# Autodesk Inventor assembly: top
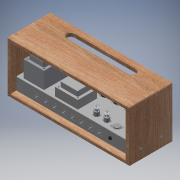
[picture p0: Inventor's stored thumbnail of the model, 180x180]
Saved by Autodesk Inventor 2016 (Build 200138000, 138)
## iProperties
Created: 2015-10-24
Part Number: top
Document SubType Name: Assembly
Designer: jeremyhale
Author: jeremyhale
## Documents named in this file (11)
- \\psf\Home\Documents\Poorhouse\git\p0001\top.iam
- \\psf\Home\Documents\Poorhouse\git\p0001\cabinet.iam
- \\psf\Home\Documents\Poorhouse\git\p0001\chassis.iam
- chassis.iam
- \\psf\Home\Documents\Poorhouse\git\p0001\cabinet-bottom.ipt
- \\psf\Home\Documents\Poorhouse\git\p0001\top\Design Accelerator\Bolted Connection6.iam
- \\psf\Home\Documents\Poorhouse\git\p0001\top\Design Accelerator\Bolted Connection7.iam
- \\psf\Home\Documents\Poorhouse\git\p0001\top\Design Accelerator\Bolted Connection8.iam
- \\psf\Home\Documents\Poorhouse\git\p0001\top\Design Accelerator\Bolted Connection9.iam
- \\psf\Home\Documents\Poorhouse\git\p0001\top\Design Accelerator\Bolted Connection10.iam
- \\psf\Home\Documents\Poorhouse\git\p0001\top\Design Accelerator\Bolted Connection11.iam
## Components (9 placed, 4 different names)
1. cabinet:1 [sub-assembly] — Flush:2, Flush:3, Flush:6, Flush:8, Flush:9, Mate:14, Mate:19, Mate:21
2. chassis:1 [sub-assembly] — Mate:1, Flush:4, Flush:5, Mate:20, Mate:22, Mate:24, Mate:26, Mate:28, Mate:30
3. cabinet-bottom:1 — Mate:1, Flush:4, Flush:5, Flush:6, Flush:8, Flush:9, Mate:14, Mate:23, Mate:25, Mate:27, Mate:29
4. Bolted Connection:5 [sub-assembly] — Mate:19, Mate:20
5. Bolted Connection:6 [sub-assembly] — Mate:21, Mate:22
6. Bolted Connection:1 [sub-assembly] — Mate:27, Mate:28
7. Bolted Connection:2 [sub-assembly] — Mate:29, Mate:30
8. Bolted Connection:3 [sub-assembly] — Mate:25, Mate:26
9. Bolted Connection:4 [sub-assembly] — Mate:23, Mate:24
## Relationships (21: Mate 14, Flush 7)
- Flush:2: cabinet:1
- Flush:3: cabinet:1
- Mate:1: chassis:1 ↔ cabinet-bottom:1
- Flush:4 (-25.4 mm): chassis:1 ↔ cabinet-bottom:1
- Flush:5: chassis:1 ↔ cabinet-bottom:1
- Flush:6: cabinet:1 ↔ cabinet-bottom:1
- Flush:8: cabinet:1 ↔ cabinet-bottom:1
- Flush:9: cabinet:1 ↔ cabinet-bottom:1
- Mate:14: cabinet:1 ↔ cabinet-bottom:1
- Mate:19: cabinet:1 ↔ Bolted Connection:5
- Mate:20: chassis:1 ↔ Bolted Connection:5
- Mate:21: cabinet:1 ↔ Bolted Connection:6
- Mate:22: chassis:1 ↔ Bolted Connection:6
- Mate:23: cabinet-bottom:1 ↔ Bolted Connection:4
- Mate:24: chassis:1 ↔ Bolted Connection:4
- Mate:25: cabinet-bottom:1 ↔ Bolted Connection:3
- Mate:26: chassis:1 ↔ Bolted Connection:3
- Mate:27: cabinet-bottom:1 ↔ Bolted Connection:1
- Mate:28: chassis:1 ↔ Bolted Connection:1
- Mate:29: cabinet-bottom:1 ↔ Bolted Connection:2
- Mate:30: chassis:1 ↔ Bolted Connection:2
